# Autodesk Inventor assembly: FineSawToothClip
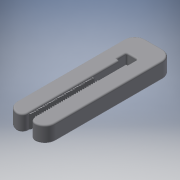
[picture p0: Inventor's stored thumbnail of the model, 180x180]
Saved by Autodesk Inventor 2016 (Build 200138000, 138)
## iProperties
Created: 2016-03-25
Part Number: FineSawToothClip
Document SubType Name: Assembly
Designer: yash
Author: yash
## Documents named in this file (3)
- C:\Users\yash\Documents\GitHub\HeadphoneBackClip\FineSawToothClip.iam
- C:\Users\yash\Documents\GitHub\HeadphoneBackClip\BaseClip.ipt
- C:\Users\yash\Documents\GitHub\HeadphoneBackClip\SawTeethFine.ipt
## Components (2 placed, 2 different names)
1. BaseClip:1 — Mate:1, Mate:2, Mate:3, Mate:4, Mate:5, Mate:6
2. SawTeethFine:1 — Mate:1, Mate:2, Mate:3, Mate:4, Mate:5, Mate:6
## Relationships (6: Mate 6)
- Mate:1: BaseClip:1 ↔ SawTeethFine:1
- Mate:2: BaseClip:1 ↔ SawTeethFine:1
- Mate:3: BaseClip:1 ↔ SawTeethFine:1
- Mate:4: BaseClip:1 ↔ SawTeethFine:1
- Mate:5: BaseClip:1 ↔ SawTeethFine:1
- Mate:6: BaseClip:1 ↔ SawTeethFine:1
